# Autodesk Inventor assembly: Fender and Igus_MIR
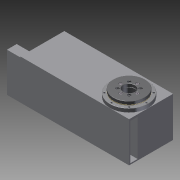
[picture p0: Inventor's stored thumbnail of the model, 180x180]
Saved by Autodesk Inventor 2015 (Build 190159000, 159)
## iProperties
Created: 2015-01-19
Part Number: Fender and Igus_MIR
Document SubType Name: Assembly
Designer: chapale16
Author: chapale16
## Documents named in this file (4)
- \\lhssvr02\Homedirs\Robotics Club\CAD Model 2015\Fender and Igus_MIR.iam
- \\lhssvr02\Homedirs\Robotics Club\CAD Model 2015\Game Components\The Tote Collector-Arms\Imported Components\PRT_01_30_1\PRT_01_30_1_MIR.iam
- \\lhssvr02\Homedirs\Robotics Club\CAD Model 2015\Bearing plate version 2.0_MIR.ipt
- \\lhssvr02\Homedirs\Robotics Club\CAD Model 2015\Fc Fender Assembly_MIR1.iam
## Components (3 placed, 3 different names)
1. PRT_01_30_1_MIR:1 [sub-assembly] — Mate:2, Mate:1, Mate:4
2. Bearing plate version 2.0_MIR:1 — Mate:2, Mate:1, Mate:3
3. Fc Fender Assembly_MIR1:1 [sub-assembly] — Mate:4, Mate:3
## Relationships (4: Mate 4)
- Mate:2: PRT_01_30_1_MIR:1 ↔ Bearing plate version 2.0_MIR:1
- Mate:1: PRT_01_30_1_MIR:1 ↔ Bearing plate version 2.0_MIR:1
- Mate:4: PRT_01_30_1_MIR:1 ↔ Fc Fender Assembly_MIR1:1
- Mate:3: Bearing plate version 2.0_MIR:1 ↔ Fc Fender Assembly_MIR1:1
